# Autodesk Inventor assembly: Servo_Shaft_2
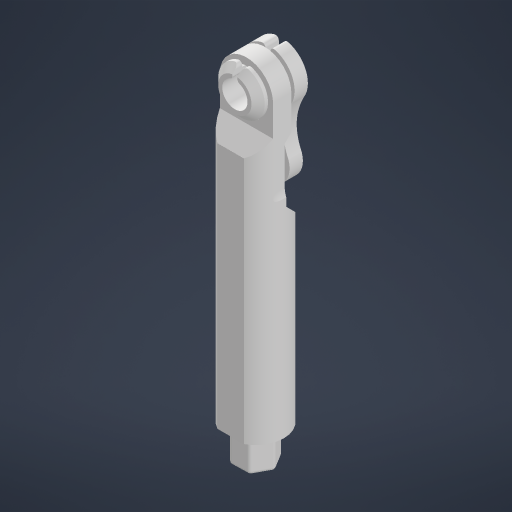
[picture p0: Inventor's stored thumbnail of the model, 512x512]
Saved by Autodesk Inventor 2024 (Build 280153000, 153)
## iProperties
Created: 2025-09-14
Part Number: Servo_Shaft_2
Document SubType Name: Assembly
Designer: kevin
Author: kevin
## Documents named in this file (3)
- C:\Users\kevin\Desktop\SeniorDesign\Servo_Shaft_2.iam
- C:\Users\kevin\Desktop\SeniorDesign\Shaft_Long.ipt
- C:\Users\kevin\Desktop\Servo_Pulley.ipt
## Components (2 placed, 2 different names)
1. Shaft_Long:1 — Mate:1, Mate:2
2. Servo_Pulley:1 — Mate:1, Mate:2
## Relationships (2: Mate 2)
- Mate:1: Shaft_Long:1 ↔ Servo_Pulley:1
- Mate:2 (1 mm): Shaft_Long:1 ↔ Servo_Pulley:1
